# Autodesk Inventor assembly: Door-Assembly-Group2
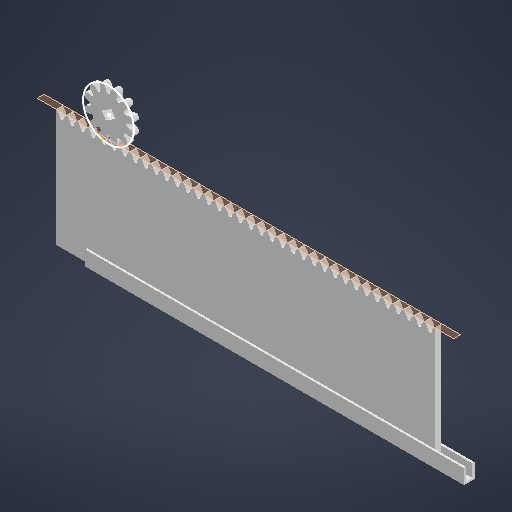
[picture p0: Inventor's stored thumbnail of the model, 512x512]
Saved by Autodesk Inventor 2026.2 (Build 302298010, 298A)
## iProperties
Created: 2026-02-27
Part Number: Door-Assembly-Group2
Document SubType Name: Assembly
Designer: ba2032
Author: ba2032
## Documents named in this file (4)
- C:\Users\bobmi\OneDrive - Heriot-Watt University\Github\System-Project-G2\mechanical\door-assembly-group2.iam
- C:\Users\bobmi\OneDrive - Heriot-Watt University\Github\System-Project-G2\mechanical\door\door-pinion-group2.ipt
- C:\Users\bobmi\OneDrive - Heriot-Watt University\Github\System-Project-G2\mechanical\door\door-group2.ipt
- C:\Users\bobmi\OneDrive - Heriot-Watt University\Github\System-Project-G2\mechanical\door\door-rail-group2.ipt
## Components (3 placed, 3 different names)
1. door-pinion-group2:1 — Mate:1, Flush:1, Flush:2, Rotation/Translation:2
2. door-group2:1 — Flush:2, Flush:3, Slider:1, Rotation/Translation:2
3. door-rail-group2:1 — Flush:4, Slider:1, Mate:2
## Relationships (8: Flush 4, Mate 2, TranslationJoint 1, RelateRotateTranslate 1)
- Mate:1: door-pinion-group2:1
- Flush:1: door-pinion-group2:1
- Flush:2: door-pinion-group2:1 ↔ door-group2:1
- Flush:3 (10.043 mm): door-group2:1
- Flush:4 (-1 mm): door-rail-group2:1
- Slider:1 [TranslationJoint]: door-group2:1 ↔ door-rail-group2:1
- Mate:2 (-10 mm): door-rail-group2:1
- Rotation/Translation:2 [RelateRotateTranslate] (60 mm): door-pinion-group2:1 ↔ door-group2:1
